# Autodesk Inventor assembly: elevator
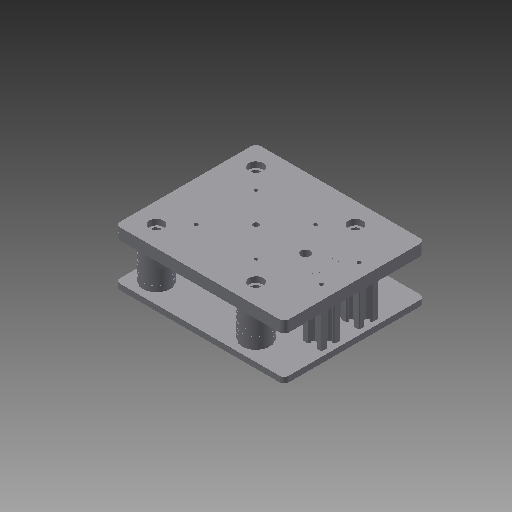
[picture p0: Inventor's stored thumbnail of the model, 512x512]
Saved by Autodesk Inventor 2019 (Build 230136000, 136)
## iProperties
Created: 2021-11-01
Part Number: elevator
Document SubType Name: Assembly
Designer: Mohamed
Author: Mohamed
## Documents named in this file (10)
- D:\mody\IndustrialLine\SortingAndStorage\Inventor\SSCARA Robot\elevator.iam
- D:\mody\IndustrialLine\SortingAndStorage\Inventor\SSCARA Robot\E_base1.ipt
- D:\mody\IndustrialLine\SortingAndStorage\Inventor\SSCARA Robot\e_guid nut.ipt
- D:\mody\IndustrialLine\SortingAndStorage\Inventor\SSCARA Robot\E_base2.ipt
- D:\mody\IndustrialLine\SortingAndStorage\Inventor\SSCARA Robot\e_linear bearing 10mm.ipt
- D:\mody\IndustrialLine\SortingAndStorage\Inventor\SSCARA Robot\e_support 1.ipt
- D:\mody\IndustrialLine\SortingAndStorage\Inventor\SSCARA Robot\e_V-Slot 20x20x40Linear Rail.ipt
- D:\mody\IndustrialLine\SortingAndStorage\Inventor\SSCARA Robot\e_support 2.ipt
- D:\mody\IndustrialLine\SortingAndStorage\Inventor\SSCARA Robot\e_spacer 4mm.ipt
- D:\mody\IndustrialLine\SortingAndStorage\Inventor\SSCARA Robot\e_spacer 6mm.ipt
## Components (30 placed, 9 different names)
1. E_base1:1 — Mate:1, Mate:2, Mate:3, Mate:4, Mate:5, Mate:6, Mate:7, Mate:8, Mate:10, Mate:17, Mate:24, Mate:25, Mate:26, Mate:27, Mate:28, Mate:29
2. e_guid nut:1 — Mate:1, Mate:2
3. E_base2:1 — Mate:3, Mate:4, Mate:5, Mate:6, Mate:9, Mate:11, Mate:12, Mate:13, Mate:14, Flush:2
4. e_linear bearing 10mm:1 — Mate:8, Mate:13, Mate:56
5. e_linear bearing 10mm:2 — Mate:9, Mate:11, Mate:59
6. e_linear bearing 10mm:3 — Mate:10, Mate:12, Mate:15, Mate:18, Mate:22, Mate:58
7. e_linear bearing 10mm:4 — Mate:7, Mate:14, Mate:16, Mate:19, Mate:21, Mate:57
8. e_support 1:1 — Mate:15, Mate:16, Mate:17, Mate:20
9. e_support 1:2 — Mate:18, Mate:19, Mate:20, Mate:23
10. e_support 1:3 — Mate:21, Mate:22, Mate:23, Mate:60, Mate:61, Mate:62, Mate:63
11. e_V-Slot 20x20x40Linear Rail:1 — Mate:24, Mate:27, Flush:1, Mate:31
12. e_V-Slot 20x20x40Linear Rail:2 — Mate:25, Mate:26, Flush:1, Mate:30
13. e_support 2:1 — Flush:2, Mate:28, Mate:29, Flush:3
14. E_base1:2 — Flush:3, Mate:30, Mate:31
15. e_spacer 4mm:1 — Mate:33, Mate:35, Mate:56, Mate:62
16. e_spacer 6mm:1 — Mate:32, Mate:34, Mate:35, Mate:36
17. e_spacer 6mm:2 — Mate:32, Mate:33, Mate:34, Mate:37
18. e_spacer 6mm:3 — Mate:36, Mate:37
19. e_spacer 4mm:2 — Mate:58, Mate:61
20. e_spacer 6mm:4
21. e_spacer 6mm:5
22. e_spacer 6mm:6
23. e_spacer 4mm:3 — Mate:59, Mate:60
24. e_spacer 6mm:7
25. e_spacer 6mm:8
26. e_spacer 6mm:9
27. e_spacer 4mm:4 — Mate:57, Mate:63
28. e_spacer 6mm:10
29. e_spacer 6mm:11
30. e_spacer 6mm:12
## Relationships (66: Mate 63, Flush 3)
- Mate:1: E_base1:1 ↔ e_guid nut:1
- Mate:2: E_base1:1 ↔ e_guid nut:1
- Mate:3: E_base1:1 ↔ E_base2:1
- Mate:4: E_base1:1 ↔ E_base2:1
- Mate:5: E_base1:1 ↔ E_base2:1
- Mate:6: E_base1:1 ↔ E_base2:1
- Mate:7: E_base1:1 ↔ e_linear bearing 10mm:4
- Mate:8: E_base1:1 ↔ e_linear bearing 10mm:1
- Mate:9: E_base2:1 ↔ e_linear bearing 10mm:2
- Mate:10: E_base1:1 ↔ e_linear bearing 10mm:3
- Mate:11: E_base2:1 ↔ e_linear bearing 10mm:2
- Mate:12: E_base2:1 ↔ e_linear bearing 10mm:3
- Mate:13: E_base2:1 ↔ e_linear bearing 10mm:1
- Mate:14: E_base2:1 ↔ e_linear bearing 10mm:4
- Mate:15: e_linear bearing 10mm:3 ↔ e_support 1:1
- Mate:16: e_linear bearing 10mm:4 ↔ e_support 1:1
- Mate:17: E_base1:1 ↔ e_support 1:1
- Mate:18: e_linear bearing 10mm:3 ↔ e_support 1:2
- Mate:19: e_linear bearing 10mm:4 ↔ e_support 1:2
- Mate:20: e_support 1:1 ↔ e_support 1:2
- Mate:21: e_linear bearing 10mm:4 ↔ e_support 1:3
- Mate:22: e_linear bearing 10mm:3 ↔ e_support 1:3
- Mate:23: e_support 1:2 ↔ e_support 1:3
- Mate:24: E_base1:1 ↔ e_V-Slot 20x20x40Linear Rail:1
- Mate:25: E_base1:1 ↔ e_V-Slot 20x20x40Linear Rail:2
- Mate:26: E_base1:1 ↔ e_V-Slot 20x20x40Linear Rail:2
- Mate:27: E_base1:1 ↔ e_V-Slot 20x20x40Linear Rail:1
- Flush:1: e_V-Slot 20x20x40Linear Rail:1 ↔ e_V-Slot 20x20x40Linear Rail:2
- Flush:2: E_base2:1 ↔ e_support 2:1
- Mate:28: E_base1:1 ↔ e_support 2:1
- Mate:29: E_base1:1 ↔ e_support 2:1
- Flush:3: e_support 2:1 ↔ E_base1:2
- Mate:30: e_V-Slot 20x20x40Linear Rail:2 ↔ E_base1:2
- Mate:31: e_V-Slot 20x20x40Linear Rail:1 ↔ E_base1:2
- Mate:32: e_spacer 6mm:1 ↔ e_spacer 6mm:2
- Mate:33: e_spacer 4mm:1 ↔ e_spacer 6mm:2
- Mate:34: e_spacer 6mm:1 ↔ e_spacer 6mm:2
- Mate:35: e_spacer 4mm:1 ↔ e_spacer 6mm:1
- Mate:36: e_spacer 6mm:1 ↔ e_spacer 6mm:3
- Mate:37: e_spacer 6mm:2 ↔ e_spacer 6mm:3
- [Mate]: e_spacer 6mm:4 ↔ e_spacer 6mm:5
- [Mate]: e_spacer 4mm:2 ↔ e_spacer 6mm:5
- [Mate]: e_spacer 6mm:4 ↔ e_spacer 6mm:5
- [Mate]: e_spacer 4mm:2 ↔ e_spacer 6mm:4
- [Mate]: e_spacer 6mm:4 ↔ e_spacer 6mm:6
- [Mate]: e_spacer 6mm:5 ↔ e_spacer 6mm:6
- [Mate]: e_spacer 6mm:7 ↔ e_spacer 6mm:8
- [Mate]: e_spacer 4mm:3 ↔ e_spacer 6mm:8
- [Mate]: e_spacer 6mm:7 ↔ e_spacer 6mm:8
- [Mate]: e_spacer 4mm:3 ↔ e_spacer 6mm:7
- [Mate]: e_spacer 6mm:7 ↔ e_spacer 6mm:9
- [Mate]: e_spacer 6mm:8 ↔ e_spacer 6mm:9
- [Mate]: e_spacer 6mm:10 ↔ e_spacer 6mm:11
- [Mate]: e_spacer 4mm:4 ↔ e_spacer 6mm:11
- [Mate]: e_spacer 6mm:10 ↔ e_spacer 6mm:11
- [Mate]: e_spacer 4mm:4 ↔ e_spacer 6mm:10
- [Mate]: e_spacer 6mm:10 ↔ e_spacer 6mm:12
- [Mate]: e_spacer 6mm:11 ↔ e_spacer 6mm:12
- Mate:56: e_linear bearing 10mm:1 ↔ e_spacer 4mm:1
- Mate:57: e_linear bearing 10mm:4 ↔ e_spacer 4mm:4
- Mate:58: e_linear bearing 10mm:3 ↔ e_spacer 4mm:2
- Mate:59: e_linear bearing 10mm:2 ↔ e_spacer 4mm:3
- Mate:60: e_support 1:3 ↔ e_spacer 4mm:3
- Mate:61: e_support 1:3 ↔ e_spacer 4mm:2
- Mate:62: e_support 1:3 ↔ e_spacer 4mm:1
- Mate:63: e_support 1:3 ↔ e_spacer 4mm:4
## Named parameters: d49_d39 = 0 mm, d50_d40 = 0 mm, d51_d41 = 0 mm, d52_d42 = 0 mm, d53_d43 = 0 mm, d54_d44 = 0 mm, d55_d39 = 0 mm, d56_d40 = 0 mm, d57_d41 = 0 mm, d58_d42 = 0 mm, d59_d43 = 0 mm, d60_d44 = 0 mm, d61_d39 = 0 mm, d62_d40 = 0 mm, d63_d41 = 0 mm, d64_d42 = 0 mm, d65_d43 = 0 mm, d66_d44 = 0 mm
